# Autodesk Inventor assembly: Attacker_v1
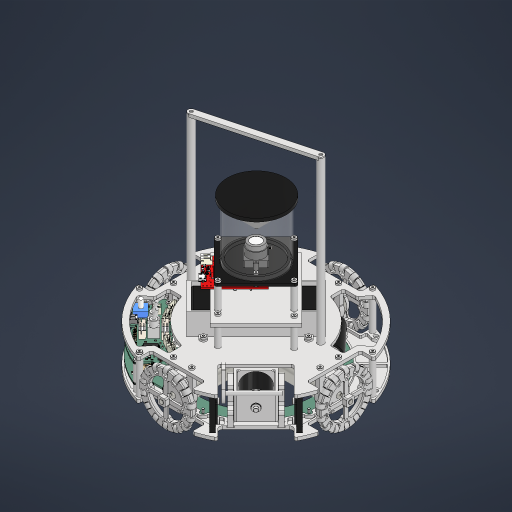
[picture p0: Inventor's stored thumbnail of the model, 512x512]
Saved by Autodesk Inventor 2024.2 (Build 282272000, 272)
## iProperties
Created: 2023-12-21
Part Number: Attacker_v1
Document SubType Name: Assembly
Designer: Hanaoka
Author: Hanaoka
## Documents named in this file (19)
- G:\共有ドライブ\reRo\05_個人\hanaoka\inventor\Attacker_v1.iam
- G:\共有ドライブ\reRo\05_個人\hanaoka\inventor\DriveUnit\DriveUnit.iam
- G:\共有ドライブ\reRo\05_個人\hanaoka\inventor\BasePlate.ipt
- G:\共有ドライブ\reRo\05_個人\hanaoka\inventor\Spacer\Spacer_M2.6x35.ipt
- G:\共有ドライブ\reRo\05_個人\hanaoka\inventor\Ball.ipt
- G:\共有ドライブ\reRo\05_個人\hanaoka\inventor\KickerUnit\KickerUnit.iam
- G:\共有ドライブ\reRo\05_個人\hanaoka\inventor\SecondPlate.ipt
- G:\共有ドライブ\reRo\05_個人\hanaoka\inventor\CameraUnit\CameraUnit.iam
- G:\共有ドライブ\reRo\05_個人\hanaoka\inventor\BatteryUnit\BatteryUnit.iam
- G:\共有ドライブ\reRo\05_個人\hanaoka\inventor\DribblerUnit\DribblerUnit.iam
- G:\共有ドライブ\reRo\05_個人\hanaoka\inventor\Spacer\Spacer_M2.6x25.ipt
- G:\共有ドライブ\reRo\05_個人\hanaoka\inventor\ThirdPlate.ipt
- G:\共有ドライブ\reRo\05_個人\hanaoka\inventor\HandleUnit\HandleUnit.iam
- G:\共有ドライブ\reRo\05_個人\hanaoka\inventor\BallSensorUnit\BallSensorUnit.iam
- G:\共有ドライブ\reRo\05_個人\hanaoka\inventor\Screw\M2.6x8\M2.6x8.ipt
- G:\共有ドライブ\reRo\05_個人\hanaoka\inventor\PCBs\PCBsUnit.iam
- G:\共有ドライブ\reRo\05_個人\hanaoka\inventor\PCBs\LineSensorUnit.iam
- G:\共有ドライブ\reRo\05_個人\hanaoka\inventor\PCBs\KickerPCB_Unit.iam
- G:\共有ドライブ\reRo\05_個人\hanaoka\inventor\PCBs\CapacitorUnit.iam
## Components (42 placed, 18 different names)
1. BasePlate:1 — メイト:1, メイト:2, メイト:3, メイト:4, 挿入:1, メイト:5, メイト:6, メイト:7, メイト:8, メイト:9, メイト:10, メイト:11, メイト:12, メイト:13, メイト:14, メイト:15, メイト:16, 挿入:2, 挿入:3, 挿入:4, メイト:25, メイト:26, メイト:27, メイト:28, メイト:29, メイト:30, メイト:42, メイト:43, メイト:44, メイト:45, メイト:46, メイト:47, メイト:48, メイト:49, メイト:50, メイト:51, メイト:52, メイト:53, 挿入:9, 挿入:10, 挿入:11, 挿入:12, 挿入:29, 挿入:30, メイト:54, メイト:55, メイト:56, 挿入:33, 挿入:34
2. DriveUnit:1 [sub-assembly] — メイト:2, メイト:3, メイト:4
3. DriveUnit:2 [sub-assembly] — メイト:7, メイト:10, メイト:11
4. DriveUnit:3 [sub-assembly] — メイト:6, メイト:8, メイト:9
5. DriveUnit:4 [sub-assembly] — メイト:5, メイト:12, メイト:13
6. Spacer_M2.6x35:1 — 挿入:1
7. Spacer_M2.6x35:2 — メイト:16, 挿入:3, フラッシュ:5
8. Spacer_M2.6x35:3 — メイト:15, 挿入:4
9. Spacer_M2.6x35:4 — メイト:14, 挿入:2
10. Ball:1
11. KickerUnit:1 [sub-assembly] — メイト:25, メイト:26, メイト:27
12. KickerUnit:2 [sub-assembly] — メイト:28, メイト:29, メイト:30
13. SecondPlate:1 — フラッシュ:5, メイト:31, メイト:32, メイト:33, メイト:34, メイト:35, メイト:36, メイト:37, メイト:38, メイト:39, メイト:40, メイト:41, 挿入:25, 挿入:26, 挿入:27, 挿入:28, 挿入:35, 挿入:36
14. BatteryUnit:1 [sub-assembly] — メイト:31, メイト:32, メイト:33
15. DribblerUnit:1 [sub-assembly]
16. Spacer_M2.6x25:1 — メイト:34, メイト:38, フラッシュ:6
17. Spacer_M2.6x25:2 — メイト:37, メイト:41
18. Spacer_M2.6x25:3 — メイト:35, メイト:39
19. Spacer_M2.6x25:4 — メイト:36, メイト:40
20. ThirdPlate:1 — フラッシュ:6, 挿入:13, 挿入:14, 挿入:15, 挿入:16, 挿入:31, 挿入:37
21. CameraUnit:2 [sub-assembly] — 挿入:31, 挿入:37
22. HandleUnit:1 [sub-assembly] — 挿入:35, 挿入:36
23. BallSensorUnit:1 [sub-assembly] — メイト:43, メイト:51, メイト:53
24. BallSensorUnit:2 [sub-assembly] — メイト:45, メイト:46, メイト:47
25. BallSensorUnit:3 [sub-assembly] — メイト:44, メイト:48, メイト:49
26. BallSensorUnit:4 [sub-assembly] — メイト:42, メイト:50, メイト:52
27. M2.6x8:1 — 挿入:9
28. M2.6x8:2 — 挿入:10
29. M2.6x8:3 — 挿入:12
30. M2.6x8:4 — 挿入:11
31. M2.6x8:5 — 挿入:14
32. M2.6x8:6 — 挿入:13
33. M2.6x8:7 — 挿入:15
34. M2.6x8:8 — 挿入:16
35. M2.6x8:9 — 挿入:27
36. M2.6x8:10 — 挿入:28
37. M2.6x8:11 — 挿入:26
38. M2.6x8:12 — 挿入:25
39. PCBsUnit:1 [sub-assembly] — 挿入:29, 挿入:30
40. LineSensorUnit:1 [sub-assembly] — メイト:54, メイト:55, メイト:56
41. KickerPCB_Unit:1 [sub-assembly] — 挿入:33, 挿入:34
42. CapacitorUnit:1 [sub-assembly]
## Relationships (74: Mate 48, Insert 24, Flush 2)
- メイト:1 [Mate]: BasePlate:1
- メイト:2 [Mate]: BasePlate:1 ↔ DriveUnit:1
- メイト:3 [Mate]: BasePlate:1 ↔ DriveUnit:1
- メイト:4 [Mate]: BasePlate:1 ↔ DriveUnit:1
- 挿入:1 [Insert]: BasePlate:1 ↔ Spacer_M2.6x35:1
- メイト:5 [Mate]: BasePlate:1 ↔ DriveUnit:4
- メイト:6 [Mate]: BasePlate:1 ↔ DriveUnit:3
- メイト:7 [Mate]: BasePlate:1 ↔ DriveUnit:2
- メイト:8 [Mate]: BasePlate:1 ↔ DriveUnit:3
- メイト:9 [Mate]: BasePlate:1 ↔ DriveUnit:3
- メイト:10 [Mate]: BasePlate:1 ↔ DriveUnit:2
- メイト:11 [Mate]: BasePlate:1 ↔ DriveUnit:2
- メイト:12 [Mate]: BasePlate:1 ↔ DriveUnit:4
- メイト:13 [Mate]: BasePlate:1 ↔ DriveUnit:4
- メイト:14 [Mate]: BasePlate:1 ↔ Spacer_M2.6x35:4
- メイト:15 [Mate]: BasePlate:1 ↔ Spacer_M2.6x35:3
- メイト:16 [Mate]: BasePlate:1 ↔ Spacer_M2.6x35:2
- 挿入:2 [Insert]: BasePlate:1 ↔ Spacer_M2.6x35:4
- 挿入:3 [Insert]: BasePlate:1 ↔ Spacer_M2.6x35:2
- 挿入:4 [Insert]: BasePlate:1 ↔ Spacer_M2.6x35:3
- メイト:25 [Mate]: BasePlate:1 ↔ KickerUnit:1
- メイト:26 [Mate]: BasePlate:1 ↔ KickerUnit:1
- メイト:27 [Mate]: BasePlate:1 ↔ KickerUnit:1
- メイト:28 [Mate]: BasePlate:1 ↔ KickerUnit:2
- メイト:29 [Mate]: BasePlate:1 ↔ KickerUnit:2
- メイト:30 [Mate]: BasePlate:1 ↔ KickerUnit:2
- フラッシュ:5 [Flush]: Spacer_M2.6x35:2 ↔ SecondPlate:1
- メイト:31 [Mate]: SecondPlate:1 ↔ BatteryUnit:1
- メイト:32 [Mate]: SecondPlate:1 ↔ BatteryUnit:1
- メイト:33 [Mate]: SecondPlate:1 ↔ BatteryUnit:1
- メイト:34 [Mate]: SecondPlate:1 ↔ Spacer_M2.6x25:1
- メイト:35 [Mate]: SecondPlate:1 ↔ Spacer_M2.6x25:3
- メイト:36 [Mate]: SecondPlate:1 ↔ Spacer_M2.6x25:4
- メイト:37 [Mate]: SecondPlate:1 ↔ Spacer_M2.6x25:2
- メイト:38 [Mate]: SecondPlate:1 ↔ Spacer_M2.6x25:1
- メイト:39 [Mate]: SecondPlate:1 ↔ Spacer_M2.6x25:3
- メイト:40 [Mate]: SecondPlate:1 ↔ Spacer_M2.6x25:4
- メイト:41 [Mate]: SecondPlate:1 ↔ Spacer_M2.6x25:2
- フラッシュ:6 [Flush]: Spacer_M2.6x25:1 ↔ ThirdPlate:1
- メイト:42 [Mate]: BasePlate:1 ↔ BallSensorUnit:4
- メイト:43 [Mate]: BasePlate:1 ↔ BallSensorUnit:1
- メイト:44 [Mate]: BasePlate:1 ↔ BallSensorUnit:3
- メイト:45 [Mate]: BasePlate:1 ↔ BallSensorUnit:2
- メイト:46 [Mate]: BasePlate:1 ↔ BallSensorUnit:2
- メイト:47 [Mate]: BasePlate:1 ↔ BallSensorUnit:2
- メイト:48 [Mate]: BasePlate:1 ↔ BallSensorUnit:3
- メイト:49 [Mate]: BasePlate:1 ↔ BallSensorUnit:3
- メイト:50 [Mate]: BasePlate:1 ↔ BallSensorUnit:4
- メイト:51 [Mate]: BasePlate:1 ↔ BallSensorUnit:1
- メイト:52 [Mate]: BasePlate:1 ↔ BallSensorUnit:4
- メイト:53 [Mate]: BasePlate:1 ↔ BallSensorUnit:1
- 挿入:9 [Insert]: BasePlate:1 ↔ M2.6x8:1
- 挿入:10 [Insert]: BasePlate:1 ↔ M2.6x8:2
- 挿入:11 [Insert]: BasePlate:1 ↔ M2.6x8:4
- 挿入:12 [Insert]: BasePlate:1 ↔ M2.6x8:3
- 挿入:13 [Insert]: ThirdPlate:1 ↔ M2.6x8:6
- 挿入:14 [Insert]: ThirdPlate:1 ↔ M2.6x8:5
- 挿入:15 [Insert]: ThirdPlate:1 ↔ M2.6x8:7
- 挿入:16 [Insert]: ThirdPlate:1 ↔ M2.6x8:8
- 挿入:25 [Insert]: SecondPlate:1 ↔ M2.6x8:12
- 挿入:26 [Insert]: SecondPlate:1 ↔ M2.6x8:11
- 挿入:27 [Insert]: SecondPlate:1 ↔ M2.6x8:9
- 挿入:28 [Insert]: SecondPlate:1 ↔ M2.6x8:10
- 挿入:29 [Insert]: BasePlate:1 ↔ PCBsUnit:1
- 挿入:30 [Insert]: BasePlate:1 ↔ PCBsUnit:1
- メイト:54 [Mate]: BasePlate:1 ↔ LineSensorUnit:1
- メイト:55 [Mate]: BasePlate:1 ↔ LineSensorUnit:1
- メイト:56 [Mate]: BasePlate:1 ↔ LineSensorUnit:1
- 挿入:31 [Insert]: ThirdPlate:1 ↔ CameraUnit:2
- 挿入:33 [Insert]: BasePlate:1 ↔ KickerPCB_Unit:1
- 挿入:34 [Insert]: BasePlate:1 ↔ KickerPCB_Unit:1
- 挿入:35 [Insert]: SecondPlate:1 ↔ HandleUnit:1
- 挿入:36 [Insert]: SecondPlate:1 ↔ HandleUnit:1
- 挿入:37 [Insert]: ThirdPlate:1 ↔ CameraUnit:2
